# Autodesk Inventor assembly: left_arm_MIR
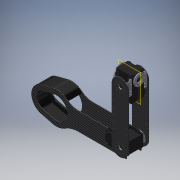
[picture p0: Inventor's stored thumbnail of the model, 180x180]
Saved by Autodesk Inventor 2018 (Build 220112000, 112)
## iProperties
Created: 2018-11-27
Part Number: left_arm_MIR
Document SubType Name: Assembly
Designer: jaspe
Author: bitbots
## Documents named in this file (6)
- C:\Users\jaspe\bitbots_hardware\wolfgang\assembly\arms\right_arm.iam
- C:\Users\jaspe\bitbots_hardware\wolfgang\assembly\arms\forearm_MIR.ipt
- C:\Users\jaspe\bitbots_hardware\wolfgang\assembly\motors\MX64\Mx64_with_bearing_MIR1.iam
- C:\Users\jaspe\bitbots_hardware\wolfgang\assembly\arms\hand_MIR.ipt
- C:\Users\jaspe\bitbots_hardware\wolfgang\assembly\arms\upperarm_MIR.ipt
- C:\Users\jaspe\bitbots_hardware\wolfgang\assembly\arms\connector_shoulder_MIR.ipt
## Components (9 placed, 5 different names)
1. forearm_MIR:1 — Mate:3, Mate:2, Mate:1, Mate:10
2. forearm_MIR:2 — Mate:6, Mate:5, Mate:4, Mate:9, Mate:8, Mate:7
3. Mx64_with_bearing_MIR1:1 [sub-assembly] — Mate:6, Mate:5, Mate:4, Mate:3, Mate:2, Mate:1, Mate:15, Mate:14, Mate:13, Mate:12, Mate:11
4. hand_MIR:1 — Mate:10, Mate:9, Mate:8, Mate:7
5. upperarm_MIR:1 — Mate:15, Mate:14, Mate:25
6. upperarm_MIR:2 — Mate:13, Mate:12, Mate:11, Mate:24, Mate:23, Mate:22
7. Mx64_with_bearing_MIR1:2 [sub-assembly] — Mate:21, Mate:20, Mate:19, Mate:18, Mate:17, Mate:16, Flush:1
8. connector_shoulder_MIR:1 — Mate:24, Mate:23, Mate:22, Mate:21, Mate:20, Mate:19
9. connector_shoulder_MIR:2 — Mate:25, Mate:18, Mate:17, Mate:16
## Relationships (26: Mate 25, Flush 1)
- Mate:6: forearm_MIR:2 ↔ Mx64_with_bearing_MIR1:1
- Mate:5: forearm_MIR:2 ↔ Mx64_with_bearing_MIR1:1
- Mate:4: forearm_MIR:2 ↔ Mx64_with_bearing_MIR1:1
- Mate:3: forearm_MIR:1 ↔ Mx64_with_bearing_MIR1:1
- Mate:2: forearm_MIR:1 ↔ Mx64_with_bearing_MIR1:1
- Mate:1: forearm_MIR:1 ↔ Mx64_with_bearing_MIR1:1
- Mate:10: forearm_MIR:1 ↔ hand_MIR:1
- Mate:9: forearm_MIR:2 ↔ hand_MIR:1
- Mate:8: forearm_MIR:2 ↔ hand_MIR:1
- Mate:7: forearm_MIR:2 ↔ hand_MIR:1
- Mate:15: Mx64_with_bearing_MIR1:1 ↔ upperarm_MIR:1
- Mate:14: Mx64_with_bearing_MIR1:1 ↔ upperarm_MIR:1
- Mate:13: Mx64_with_bearing_MIR1:1 ↔ upperarm_MIR:2
- Mate:12: Mx64_with_bearing_MIR1:1 ↔ upperarm_MIR:2
- Mate:11: Mx64_with_bearing_MIR1:1 ↔ upperarm_MIR:2
- Mate:24: upperarm_MIR:2 ↔ connector_shoulder_MIR:1
- Mate:23: upperarm_MIR:2 ↔ connector_shoulder_MIR:1
- Mate:22: upperarm_MIR:2 ↔ connector_shoulder_MIR:1
- Mate:21: Mx64_with_bearing_MIR1:2 ↔ connector_shoulder_MIR:1
- Mate:20: Mx64_with_bearing_MIR1:2 ↔ connector_shoulder_MIR:1
- Mate:19: Mx64_with_bearing_MIR1:2 ↔ connector_shoulder_MIR:1
- Mate:25: upperarm_MIR:1 ↔ connector_shoulder_MIR:2
- Mate:18: Mx64_with_bearing_MIR1:2 ↔ connector_shoulder_MIR:2
- Mate:17: Mx64_with_bearing_MIR1:2 ↔ connector_shoulder_MIR:2
- Mate:16: Mx64_with_bearing_MIR1:2 ↔ connector_shoulder_MIR:2
- Flush:1 (-14.5 mm): Mx64_with_bearing_MIR1:2
